# Autodesk Inventor assembly: 基本構造距離センサ1セット配置
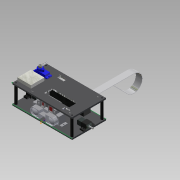
[picture p0: Inventor's stored thumbnail of the model, 180x180]
Saved by Autodesk Inventor 2017 (Build 210142000, 142)
## iProperties
Part Number: 基本構造距離センサ1セット配置
Material: 一般
Document SubType Name: Assembly
Designer: HISAAKI
Author: HISAAKI
## Documents named in this file (18)
- C:\Users\HISAAKI\Documents\LYNCS\CanSat\2017種子島\cansat-structure\基本構造距離センサ1セット配置.iam
- C:\Users\HISAAKI\Documents\LYNCS\CanSat\2017種子島\cansat-structure\基本板.ipt
- C:\Users\HISAAKI\Documents\LYNCS\CanSat\2017種子島\cansat-structure\既成部品\ブラケット.ipt
- C:\Users\HISAAKI\Documents\LYNCS\CanSat\2017種子島\cansat-structure\既成部品\モータ.ipt
- C:\Users\HISAAKI\Documents\LYNCS\CanSat\2017種子島\cansat-structure\ハブver1.1.ipt
- C:\Users\HISAAKI\Documents\LYNCS\CanSat\2017種子島\cansat-structure\タイヤスポンジ部分.ipt
- C:\Users\HISAAKI\Documents\LYNCS\CanSat\2017種子島\cansat-structure\基本板上.ipt
- C:\Users\HISAAKI\Documents\LYNCS\CanSat\2017種子島\cansat-structure\既成部品\スペーサ.ipt
- C:\Users\HISAAKI\Documents\LYNCS\CanSat\2017種子島\cansat-structure\既成部品\GPSユニット.ipt
- C:\Users\HISAAKI\Documents\LYNCS\CanSat\2017種子島\cansat-structure\基板.ipt
- C:\Users\HISAAKI\Documents\LYNCS\CanSat\2017種子島\cansat-structure\スペーサ5mm.ipt
- C:\Users\HISAAKI\Documents\LYNCS\CanSat\2017種子島\cansat-structure\タイヤプラ板部分.ipt
- C:\Users\HISAAKI\Documents\LYNCS\CanSat\2017種子島\cansat-structure\スタビライザ.ipt
- C:\Users\HISAAKI\Documents\LYNCS\CanSat\2017種子島\cansat-structure\リポ電池黒.ipt
- C:\Users\HISAAKI\Documents\LYNCS\CanSat\2017種子島\cansat-structure\センサ1セット.iam
- C:\Users\HISAAKI\Documents\LYNCS\CanSat\2017種子島\cansat-structure\mbed_NXP_LPC1768.ipt
- C:\Users\HISAAKI\Documents\LYNCS\CanSat\2017種子島\cansat-structure\XBeeProS1.ipt
- C:\Users\HISAAKI\Documents\LYNCS\CanSat\2017種子島\cansat-structure\Tower Pro 9g Micro Servo SG90.ipt
## Components (29 placed, 17 different names)
1. 基本板:1 — フラッシュ:1, フラッシュ:2, メイト:20, メイト:21, メイト:23, メイト:24, メイト:25, メイト:26, メイト:27, メイト:28, メイト:29, メイト:30, メイト:35, メイト:36, メイト:37, メイト:38, メイト:39, メイト:40, メイト:77, メイト:85, メイト:86, メイト:87, メイト:91, フラッシュ:21, フラッシュ:22, メイト:92, メイト:93, フラッシュ:23
2. モータ:1 — フラッシュ:2, メイト:13, メイト:14, メイト:41, メイト:43
3. モータ:2 — フラッシュ:1, メイト:11, メイト:12, メイト:42, メイト:44
4. ハブver1.1:1 — メイト:11, メイト:12, メイト:17, メイト:18
5. ハブver1.1:2 — メイト:13, メイト:14, メイト:15, メイト:16
6. タイヤスポンジ部分:1 — メイト:15, メイト:16, メイト:62, メイト:63
7. タイヤスポンジ部分:2 — メイト:17, メイト:18, メイト:64, メイト:65
8. 基本板上:1 — メイト:20, メイト:21, メイト:31, メイト:32, フラッシュ:5, メイト:47, メイト:48, メイト:49, メイト:50, メイト:51, メイト:52, メイト:53, メイト:54, メイト:96, メイト:97
9. スペーサ:1 — メイト:23, メイト:29
10. スペーサ:2 — メイト:25, メイト:28
11. スペーサ:3 — メイト:24, メイト:30, メイト:31
12. スペーサ:4 — メイト:26, メイト:27
13. GPSユニット:1 — メイト:32, フラッシュ:5
14. ブラケット:1 — メイト:35, メイト:36, メイト:37, メイト:41, メイト:43
15. ブラケット:2 — メイト:38, メイト:39, メイト:40, メイト:42, メイト:44
16. スペーサ5mm:1 — メイト:47, メイト:51, メイト:58
17. スペーサ5mm:2 — メイト:50, メイト:52, メイト:57
18. スペーサ5mm:3 — メイト:48, メイト:54, メイト:55, メイト:59
19. スペーサ5mm:4 — メイト:49, メイト:53, メイト:56
20. 基板:1 — メイト:55, メイト:56, メイト:57, メイト:58, メイト:59, フラッシュ:24, メイト:94, フラッシュ:25, メイト:95, フラッシュ:26
21. タイヤプラ板部分:1 — メイト:62, メイト:63
22. タイヤプラ板部分:2 — メイト:64, メイト:65
23. スタビライザ:1 — メイト:77, メイト:85, メイト:86, メイト:87
24. リポ電池黒:1 — メイト:90, フラッシュ:19, フラッシュ:20, メイト:91, フラッシュ:21, フラッシュ:22
25. リポ電池黒:2 — メイト:90, フラッシュ:19, フラッシュ:20
26. センサ1セット:1 [sub-assembly] — メイト:92, メイト:93, フラッシュ:23
27. mbed_NXP_LPC1768:1 — フラッシュ:24, メイト:94
28. XBeeProS1:1 — フラッシュ:25, メイト:95, フラッシュ:26
29. Tower Pro 9g Micro Servo SG90:1 — メイト:96, メイト:97
## Relationships (70: Mate 59, Flush 11)
- フラッシュ:1 [Flush]: 基本板:1 ↔ モータ:2
- フラッシュ:2 [Flush]: 基本板:1 ↔ モータ:1
- メイト:11 [Mate]: モータ:2 ↔ ハブver1.1:1
- メイト:12 [Mate]: モータ:2 ↔ ハブver1.1:1
- メイト:13 [Mate]: モータ:1 ↔ ハブver1.1:2
- メイト:14 [Mate]: モータ:1 ↔ ハブver1.1:2
- メイト:15 [Mate]: ハブver1.1:2 ↔ タイヤスポンジ部分:1
- メイト:16 [Mate]: ハブver1.1:2 ↔ タイヤスポンジ部分:1
- メイト:17 [Mate]: ハブver1.1:1 ↔ タイヤスポンジ部分:2
- メイト:18 [Mate]: ハブver1.1:1 ↔ タイヤスポンジ部分:2
- メイト:20 [Mate]: 基本板:1 ↔ 基本板上:1
- メイト:21 [Mate]: 基本板:1 ↔ 基本板上:1
- メイト:23 [Mate]: 基本板:1 ↔ スペーサ:1
- メイト:24 [Mate]: 基本板:1 ↔ スペーサ:3
- メイト:25 [Mate]: 基本板:1 ↔ スペーサ:2
- メイト:26 [Mate]: 基本板:1 ↔ スペーサ:4
- メイト:27 [Mate]: 基本板:1 ↔ スペーサ:4
- メイト:28 [Mate]: 基本板:1 ↔ スペーサ:2
- メイト:29 [Mate]: 基本板:1 ↔ スペーサ:1
- メイト:30 [Mate]: 基本板:1 ↔ スペーサ:3
- メイト:31 [Mate]: 基本板上:1 ↔ スペーサ:3
- メイト:32 [Mate]: 基本板上:1 ↔ GPSユニット:1
- フラッシュ:5 [Flush] (10 mm): 基本板上:1 ↔ GPSユニット:1
- メイト:35 [Mate]: 基本板:1 ↔ ブラケット:1
- メイト:36 [Mate]: 基本板:1 ↔ ブラケット:1
- メイト:37 [Mate]: 基本板:1 ↔ ブラケット:1
- メイト:38 [Mate]: 基本板:1 ↔ ブラケット:2
- メイト:39 [Mate]: 基本板:1 ↔ ブラケット:2
- メイト:40 [Mate]: 基本板:1 ↔ ブラケット:2
- メイト:41 [Mate]: モータ:1 ↔ ブラケット:1
- メイト:42 [Mate]: モータ:2 ↔ ブラケット:2
- メイト:43 [Mate]: モータ:1 ↔ ブラケット:1
- メイト:44 [Mate]: モータ:2 ↔ ブラケット:2
- メイト:47 [Mate]: 基本板上:1 ↔ スペーサ5mm:1
- メイト:48 [Mate]: 基本板上:1 ↔ スペーサ5mm:3
- メイト:49 [Mate]: 基本板上:1 ↔ スペーサ5mm:4
- メイト:50 [Mate]: 基本板上:1 ↔ スペーサ5mm:2
- メイト:51 [Mate]: 基本板上:1 ↔ スペーサ5mm:1
- メイト:52 [Mate]: 基本板上:1 ↔ スペーサ5mm:2
- メイト:53 [Mate]: 基本板上:1 ↔ スペーサ5mm:4
- メイト:54 [Mate]: 基本板上:1 ↔ スペーサ5mm:3
- メイト:55 [Mate]: スペーサ5mm:3 ↔ 基板:1
- メイト:56 [Mate]: スペーサ5mm:4 ↔ 基板:1
- メイト:57 [Mate]: スペーサ5mm:2 ↔ 基板:1
- メイト:58 [Mate]: スペーサ5mm:1 ↔ 基板:1
- メイト:59 [Mate]: スペーサ5mm:3 ↔ 基板:1
- メイト:62 [Mate]: タイヤスポンジ部分:1 ↔ タイヤプラ板部分:1
- メイト:63 [Mate]: タイヤスポンジ部分:1 ↔ タイヤプラ板部分:1
- メイト:64 [Mate]: タイヤスポンジ部分:2 ↔ タイヤプラ板部分:2
- メイト:65 [Mate]: タイヤスポンジ部分:2 ↔ タイヤプラ板部分:2
- メイト:77 [Mate]: 基本板:1 ↔ スタビライザ:1
- メイト:85 [Mate] (-30 mm): 基本板:1 ↔ スタビライザ:1
- メイト:86 [Mate]: 基本板:1 ↔ スタビライザ:1
- メイト:87 [Mate]: 基本板:1 ↔ スタビライザ:1
- メイト:90 [Mate]: リポ電池黒:1 ↔ リポ電池黒:2
- フラッシュ:19 [Flush]: リポ電池黒:1 ↔ リポ電池黒:2
- フラッシュ:20 [Flush]: リポ電池黒:1 ↔ リポ電池黒:2
- メイト:91 [Mate]: 基本板:1 ↔ リポ電池黒:1
- フラッシュ:21 [Flush] (31 mm): 基本板:1 ↔ リポ電池黒:1
- フラッシュ:22 [Flush] (5 mm): 基本板:1 ↔ リポ電池黒:1
- メイト:92 [Mate]: 基本板:1 ↔ センサ1セット:1
- メイト:93 [Mate] (32.15 mm): 基本板:1 ↔ センサ1セット:1
- フラッシュ:23 [Flush]: 基本板:1 ↔ センサ1セット:1
- フラッシュ:24 [Flush]: 基板:1 ↔ mbed_NXP_LPC1768:1
- メイト:94 [Mate]: 基板:1 ↔ mbed_NXP_LPC1768:1
- フラッシュ:25 [Flush] (10 mm): 基板:1 ↔ XBeeProS1:1
- メイト:95 [Mate]: 基板:1 ↔ XBeeProS1:1
- フラッシュ:26 [Flush] (10 mm): 基板:1 ↔ XBeeProS1:1
- メイト:96 [Mate]: 基本板上:1 ↔ Tower Pro 9g Micro Servo SG90:1
- メイト:97 [Mate]: 基本板上:1 ↔ Tower Pro 9g Micro Servo SG90:1
